# Autodesk Inventor assembly: assembly
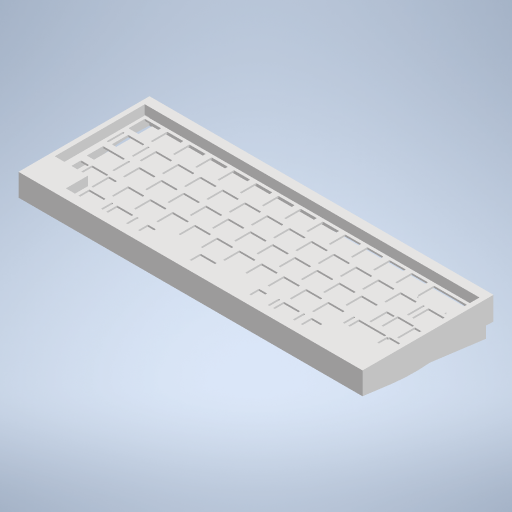
[picture p0: Inventor's stored thumbnail of the model, 512x512]
Saved by Autodesk Inventor 2024.2 (Build 282272000, 272)
## iProperties
Created: 2024-07-29
Part Number: assembly
Document SubType Name: Assembly
Designer: Eric
Author: Eric
## Documents named in this file (4)
- C:\Users\Eric\Documents\a60\CAD\assembly.iam
- C:\Users\Eric\Documents\a60\CAD\plate.ipt
- C:\Users\Eric\Documents\a60\CAD\top.ipt
- C:\Users\Eric\Documents\a60\CAD\bottom.ipt
## Components (3 placed, 3 different names)
1. plate:1 — Flush:1, Flush:2, Flush:3, Flush:4
2. top:1 — Flush:1, Flush:2
3. bottom:1 — Flush:3, Flush:4
## Relationships (4: Flush 4)
- Flush:1: plate:1 ↔ top:1
- Flush:2: plate:1 ↔ top:1
- Flush:3: plate:1 ↔ bottom:1
- Flush:4 (9.8 mm): plate:1 ↔ bottom:1
